# Autodesk Inventor assembly: ЖестьСборка
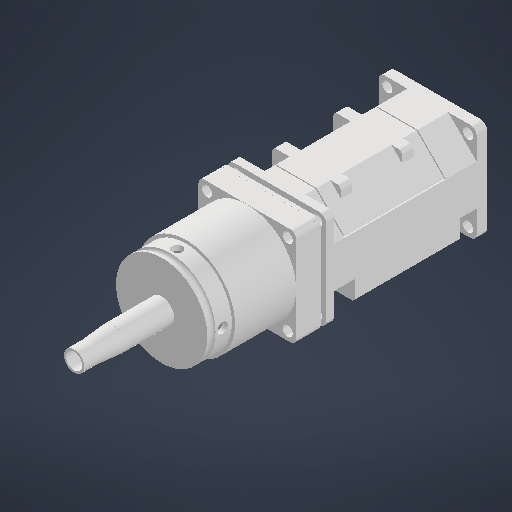
[picture p0: Inventor's stored thumbnail of the model, 512x512]
Saved by Autodesk Inventor 2026 (Build 300175000, 175)
## iProperties
Created: 2025-08-20
Part Number: ЖестьСборка
Document SubType Name: Assembly
Designer: seraf
Author: seraf
## Documents named in this file (7)
- C:\Users\seraf\Downloads\ЖестьСборка.iam
- C:\Users\seraf\OneDrive\Desktop\Печать\stl\КорпДвиг.ipt
- C:\Users\seraf\OneDrive\Desktop\Печать\stl\КрашкаКорпДвиг.ipt
- C:\Users\seraf\OneDrive\Desktop\Печать\stl\Двигатель 3115.ipt
- C:\Users\seraf\OneDrive\Desktop\Печать\stl\ПроставкаДвиг.ipt
- C:\Users\seraf\OneDrive\Desktop\Печать\stl\КорпусЕСК.ipt
- C:\Users\seraf\OneDrive\Desktop\Печать\stl\КрышкаЕСК.ipt
## Components (6 placed, 6 different names)
1. КорпДвиг:1 — Совмещение:3, Совмещение:4
2. КрашкаКорпДвиг:1 — Жесткий:1, Совмещение:1, Совмещение:3, Совмещение:4
3. Двигатель 3115:1 — Совмещение:2
4. ПроставкаДвиг:1 — Жесткий:1, Совмещение:1, Совмещение:2
5. КорпусЕСК:1 — Заподлицо:1
6. КрышкаЕСК:1 — Заподлицо:1
## Relationships (6: Mate 4, WeldJoint 1, Flush 1)
- Жесткий:1 [WeldJoint]: КрашкаКорпДвиг:1 ↔ ПроставкаДвиг:1
- Совмещение:1 [Mate]: КрашкаКорпДвиг:1 ↔ ПроставкаДвиг:1
- Совмещение:2 [Mate]: Двигатель 3115:1 ↔ ПроставкаДвиг:1
- Совмещение:3 [Mate]: КорпДвиг:1 ↔ КрашкаКорпДвиг:1
- Совмещение:4 [Mate]: КорпДвиг:1 ↔ КрашкаКорпДвиг:1
- Заподлицо:1 [Flush]: КорпусЕСК:1 ↔ КрышкаЕСК:1
## Named parameters: Finish1_Area = 46.9357
note: some values were not read from the file. Shown as the stored number, unit unknown: "Finish1_Area".
